# Autodesk Inventor assembly: アーム3
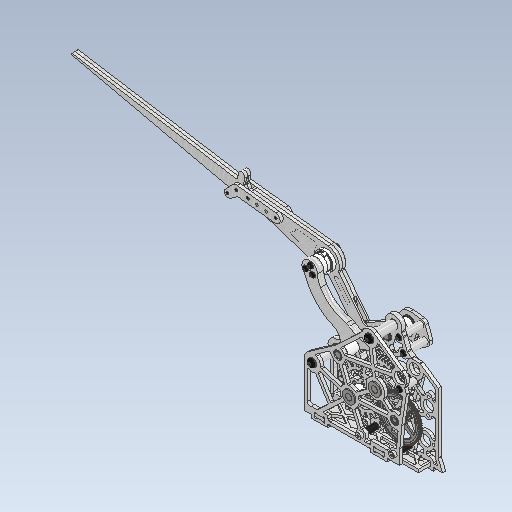
[picture p0: Inventor's stored thumbnail of the model, 512x512]
Saved by Autodesk Inventor 2020.3 (Build 243373000, 373)
## iProperties
Created: 2020-03-16
Part Number: アーム3
Document SubType Name: Assembly
Designer: aoyam
Mass: 278.23 g
Surface Area: 1026.87 cm^2
Volume: 86.6022 cm^3
Density: 3.21274 g/cm^3
Author: aoyam
## Documents named in this file (55)
- C:\Users\aoyam\Desktop\SRDC_local\Inventor\二年機\Geminiβ\腕\アーム3.iam
- C:\Users\aoyam\Desktop\SRDC_local\Inventor\二年機\Geminiβ\腕\アーム用初段.iam
- C:\Users\aoyam\Desktop\SRDC_local\Inventor\二年機\Geminiβ\腕\アーム用2段.iam
- C:\Users\aoyam\Desktop\SRDC_local\Inventor\二年機\Geminiβ\腕\アーム用3段.iam
- C:\Users\aoyam\Desktop\SRDC_local\Inventor\二年機\Geminiβ\腕\モーターマウント改.ipt
- C:\Users\aoyam\Desktop\SRDC_local\Inventor\二年機\Geminiβ\腕\アームフレーム改二.ipt
- C:\Users\aoyam\Desktop\SRDC_local\Inventor\二年機\Geminiβ\汎用部品\ベアリングHd6-D12-B4.ipt
- C:\Users\aoyam\Desktop\SRDC_local\Inventor\二年機\Geminiβ\汎用部品\ベアリングd4D8B3F.ipt
- C:\Users\aoyam\Desktop\SRDC_local\Inventor\二年機\Geminiβ\汎用部品\スペーサー中空M6L3アルミ自作.ipt
- C:\Users\aoyam\Desktop\SRDC_local\Inventor\二年機\Geminiβ\腕\アームギアフレーム最内2.ipt
- C:\Users\aoyam\Desktop\SRDC_local\Inventor\二年機\Geminiβ\腕\駆動軸.ipt
- C:\Users\aoyam\Desktop\SRDC_local\Inventor\二年機\Geminiβ\汎用部品\オイレスFd6D8L3.ipt
- C:\Users\aoyam\Desktop\SRDC_local\Inventor\二年機\Geminiβ\汎用部品\平行ピンD6L28.ipt
- C:\Users\aoyam\Desktop\SRDC_local\Inventor\二年機\Geminiβ\汎用部品\ワッシャD8d6m0.5.ipt
- C:\Users\aoyam\Desktop\SRDC_local\Inventor\二年機\Geminiβ\汎用部品\ワッシャD7d4m0.5.ipt
- C:\Users\aoyam\Desktop\SRDC_local\Inventor\二年機\Geminiβ\汎用部品\スペーサー中空M6L5樹脂.ipt
- C:\Users\aoyam\Desktop\SRDC_local\Inventor\二年機\Geminiβ\汎用部品\スペーサー中空M6L8樹脂.ipt
- C:\Users\aoyam\Desktop\SRDC_local\Inventor\二年機\Geminiβ\汎用部品\平行ピンD4L18.ipt
- C:\Users\aoyam\Desktop\SRDC_local\Inventor\二年機\Geminiβ\汎用部品\スペーサーM3L6アルミ .ipt
- C:\Users\aoyam\Desktop\SRDC_local\Inventor\二年機\Geminiβ\汎用部品\スペーサーM3L12アルミ.ipt
- C:\Users\aoyam\Desktop\SRDC_local\Inventor\二年機\Geminiβ\腕\アーム揺動節test.ipt
- C:\Users\aoyam\Desktop\SRDC_local\Inventor\二年機\Geminiβ\腕\アーム中間節test.ipt
- C:\Users\aoyam\Desktop\SRDC_local\Inventor\二年機\Geminiβ\汎用部品\オイレスFd6D8L6.ipt
- C:\Users\aoyam\Desktop\SRDC_local\Inventor\二年機\Geminiβ\腕\アームカムAL.ipt
- C:\Users\aoyam\Desktop\SRDC_local\Inventor\二年機\Geminiβ\腕\アーム中間その弐.ipt
- C:\Users\aoyam\Desktop\SRDC_local\Inventor\二年機\Geminiβ\汎用部品\ネジボタンM3L25.ipt
- C:\Users\aoyam\Desktop\SRDC_local\Inventor\二年機\Geminiβ\汎用部品\ネジボタンM3L6.ipt
- C:\Users\aoyam\Desktop\SRDC_local\Inventor\二年機\Geminiβ\汎用部品\オイレスF外径16内径14L9.ipt
- C:\Users\aoyam\Desktop\SRDC_local\Inventor\二年機\Geminiβ\汎用部品\ネジボタンM3L14.ipt
- C:\Users\aoyam\Desktop\SRDC_local\Inventor\二年機\Geminiβ\汎用部品\ネジボタンM4L6.ipt
- C:\Users\aoyam\Desktop\SRDC_local\Inventor\二年機\Geminiβ\腕\アーム揺動節抑え.ipt
- C:\Users\aoyam\Desktop\SRDC_local\Inventor\二年機\Geminiβ\汎用部品\スペーサーM3L18アルミ.ipt
- C:\Users\aoyam\Desktop\SRDC_local\Inventor\二年機\Geminiβ\腕\アーム底板.ipt
- C:\Users\aoyam\Desktop\SRDC_local\Inventor\二年機\Geminiβ\腕\アーム先端.iam
- C:\Users\aoyam\Desktop\SRDC_local\Inventor\二年機\Geminiβ\汎用部品\オイレス外径8内径6L3.ipt
- C:\Users\aoyam\Desktop\SRDC_local\Inventor\二年機\Geminiβ\汎用部品\スペーサーM3L12樹脂.ipt
- C:\Users\aoyam\Desktop\SRDC_local\Inventor\二年機\Geminiβ\汎用部品\スペーサーM3L6樹脂.ipt
- C:\Users\aoyam\Desktop\SRDC_local\Inventor\二年機\Geminiβ\汎用部品\平行ピンD6L30Dcut.ipt
- C:\Users\aoyam\Desktop\SRDC_local\Inventor\二年機\Geminiβ\汎用部品\電子機器類\RDC506018A\RDC506018A.ipt
- C:\Users\aoyam\Desktop\SRDC_local\Inventor\二年機\Geminiβ\汎用部品\ネジボタンM2L6.ipt
- C:\Users\aoyam\Desktop\SRDC_local\Inventor\二年機\Geminiβ\腕\アームカムD14.ipt
- C:\Users\aoyam\Desktop\SRDC_local\Inventor\二年機\Geminiβ\腕\アームカムD15t4.ipt
- C:\Users\aoyam\Desktop\SRDC_local\Inventor\二年機\Geminiβ\腕\アームカムFD18t4.ipt
- C:\Users\aoyam\Desktop\SRDC_local\Inventor\二年機\Geminiβ\腕\アームカムD18.ipt
- C:\Users\aoyam\Desktop\SRDC_local\Inventor\二年機\Geminiβ\汎用部品\スペーサー中空M6L2.5樹脂自作.ipt
- C:\Users\aoyam\Desktop\SRDC_local\Inventor\二年機\Geminiβ\汎用部品\スペーサーM4L21アルミ.ipt
- C:\Users\aoyam\Desktop\SRDC_local\Inventor\二年機\Geminiβ\汎用部品\ネジアルミM3L6.ipt
- C:\Users\aoyam\Desktop\SRDC_local\Inventor\二年機\Geminiβ\汎用部品\スペーサー中空M6L12樹脂.ipt
- C:\Users\aoyam\Desktop\SRDC_local\Inventor\二年機\Geminiβ\汎用部品\スペーサー中空M6L6樹脂.ipt
- C:\Users\aoyam\Desktop\SRDC_local\Inventor\二年機\インナー4層丙弐型\アーム\アーム3\AIP\FEA\d76wgh76o.fins
- C:\Users\aoyam\Desktop\SRDC_local\Inventor\二年機\インナー4層丙弐型\アーム\アーム3\AIP\FEA\d76wgh76o.fsat
- C:\Users\aoyam\Desktop\SRDC_local\Inventor\二年機\インナー4層丙弐型\アーム\アーム3\AIP\FEA\d76wgh76o.ftes
- C:\Users\aoyam\Desktop\SRDC_local\Inventor\二年機\インナー4層丙弐型\アーム\アーム3\AIP\FEA\d76wgh77k.fwiz
- C:\Users\aoyam\Desktop\SRDC_local\Inventor\二年機\インナー4層丙弐型\アーム\アーム3\AIP\FEA\d76wgh8o0.fmsh
- C:\Users\aoyam\Desktop\SRDC_local\Inventor\二年機\インナー4層丙弐型\アーム\アーム3\AIP\FEA\d76wgh8ow.fres
## Components (92 placed, 48 different names)
1. アーム用初段:1 [sub-assembly] — メイト:4, メイト:16, 挿入:204
2. アーム用2段:1 [sub-assembly] — メイト:4, メイト:6, メイト:21, メイト:27, 挿入:16, 挿入:31, 挿入:151
3. アーム用3段:1 [sub-assembly] — メイト:6, メイト:21, メイト:28, 挿入:41
4. モーターマウント改:1 — メイト:16, メイト:26, 挿入:17, メイト:30, 挿入:47, 挿入:109, メイト:73, 挿入:165, 挿入:166, 挿入:212, 挿入:213, 挿入:214, 挿入:216
5. アームフレーム改二:1 — メイト:26, メイト:27, メイト:28, 挿入:12, 挿入:13, 挿入:14, 挿入:32, 挿入:46, 挿入:135, メイト:74, 挿入:162, 挿入:208, 挿入:209, 挿入:211, 挿入:219
6. ベアリングHd6-D12-B4:1 — 挿入:13, 挿入:27
7. ベアリングd4D8B3F:1 — 挿入:12, 挿入:36, 挿入:42
8. ベアリングHd6-D12-B4:3 — 挿入:14, 挿入:28, 挿入:33
9. スペーサー中空M6L3アルミ自作:1 — 挿入:16
10. ベアリングd4D8B3F:2 — 挿入:17, 挿入:37
11. アームギアフレーム最内2:1 — メイト:30, 挿入:19, 挿入:20, 挿入:35, メイト:32, 挿入:105, 挿入:107, 挿入:110, 挿入:123, 挿入:126, メイト:69, メイト:70, メイト:71, 挿入:143, 挿入:144, 挿入:145, 挿入:150, メイト:72, 挿入:172, 挿入:173, 挿入:210, 挿入:215, 挿入:222, 角度:2, 挿入:227, 挿入:228
12. ベアリングHd6-D12-B4:4 — 挿入:19, 挿入:30, メイト:54
13. ベアリングHd6-D12-B4:5 — 挿入:20
14. 駆動軸:1 — 挿入:167, 挿入:168, 挿入:169, 挿入:201, 挿入:217, 挿入:221
15. オイレスFd6D8L3:1 — 挿入:219, 挿入:220
16. 平行ピンD6L28:1 — 挿入:27, メイト:54
17. 平行ピンD6L28:2 — 挿入:28
18. ワッシャD8d6m0.5:1 — 挿入:151
19. ワッシャD8d6m0.5:2 — 挿入:30, 挿入:39
20. ワッシャD8d6m0.5:3 — 挿入:31
21. ワッシャD8d6m0.5:4 — 挿入:32
22. ワッシャD8d6m0.5:5 — 挿入:33
23. ワッシャD8d6m0.5:7 — 挿入:35, 挿入:207
24. ワッシャD7d4m0.5:2 — 挿入:37, 挿入:205
25. ワッシャD7d4m0.5:3 — 挿入:36, 挿入:204
26. スペーサー中空M6L5樹脂:1 — 挿入:39
27. スペーサー中空M6L8樹脂:1 — 挿入:41
28. 平行ピンD4L18:1 — 挿入:42
29. スペーサーM3L12アルミ:2 — 挿入:46
30. スペーサーM3L6アルミ :2 — 挿入:47, 挿入:123
31. アーム揺動節test:1 — メイト:32, 挿入:122, 挿入:218
32. アーム中間節test:1 — 挿入:120, メイト:53, 挿入:158, 挿入:203
33. オイレスFd6D8L6:1 — 挿入:222, 挿入:223, 挿入:224
34. アームカムAL:1 — 挿入:194, 挿入:195, 挿入:196, 挿入:197, 挿入:200
35. アーム中間その弐:1 — 挿入:120, メイト:53, 挿入:122, 挿入:159, 挿入:189, メイト:84, 挿入:198
36. オイレスFd6D8L6:2 — 挿入:221, 挿入:226
37. オイレスF外径16内径14L9:1 — 挿入:197, 挿入:198, メイト:86, メイト:87
38. スペーサーM3L6アルミ :3 — 挿入:105
39. ネジボタンM3L14:1 — 挿入:107
40. ネジボタンM3L6:4 — 挿入:212
41. ネジボタンM3L6:5 — 挿入:109
42. ネジボタンM3L6:6 — 挿入:110
43. ネジボタンM3L6:7 — 挿入:211
44. ネジボタンM4L6:1 — 挿入:162
45. ネジボタンM4L6:2 — 挿入:126
46. ネジボタンM4L6:3 — 挿入:150
47. ネジボタンM4L6:4 — 挿入:135
48. オイレスFd6D8L6:3 — 挿入:225
49. アーム揺動節抑え:1 — メイト:69, メイト:70, メイト:71, 挿入:140, 挿入:141, 挿入:142, 挿入:146, 挿入:147, 挿入:148
50. スペーサーM3L18アルミ:1 — 挿入:140
51. スペーサーM3L18アルミ:2 — 挿入:141
52. スペーサーM3L18アルミ:3 — 挿入:142, 挿入:227
53. ネジボタンM3L6:16 — 挿入:143
54. ネジボタンM3L6:17 — 挿入:144
55. ネジボタンM3L6:18 — 挿入:145
56. ネジボタンM3L6:19 — 挿入:146
57. ネジボタンM3L6:20 — 挿入:147
58. ネジボタンM3L6:21 — 挿入:148
59. アーム底板:1 — メイト:72, メイト:73, メイト:74
60. アーム先端:1 [sub-assembly] — 挿入:189, メイト:84
61. オイレス外径8内径6L3:1 — 挿入:158
62. ネジボタンM3L6:22 — 挿入:159
63. スペーサーM3L12樹脂:1 — 挿入:165
64. スペーサーM3L12樹脂:2 — 挿入:166
65. スペーサーM3L6樹脂:1 — 挿入:228
66. ネジボタンM3L25:1 — 挿入:168, 挿入:196
67. ネジボタンM3L25:2 — 挿入:167, 挿入:195
68. ネジボタンM3L25:3 — 挿入:169, 挿入:194, メイト:88
69. 平行ピンD6L30Dcut:1 — 挿入:171, 角度:1, 挿入:226
70. RDC506018A:1 — 挿入:171, 角度:1, 角度:2
71. ネジボタンM2L6:1 — 挿入:172
72. ネジボタンM2L6:2 — 挿入:173
73. 平行ピンD6L28:3 — 挿入:224
74. アームカムD14:1 — 挿入:199, メイト:85, メイト:86, 挿入:202
75. アームカムD14:2 — 挿入:199, メイト:85, 挿入:200
76. アームカムD15t4:1 — 挿入:201, メイト:87
77. アームカムFD18t4:1 — 挿入:202, メイト:88
78. アームカムD18:1 — 挿入:203
79. スペーサー中空M6L2.5樹脂自作:1 — 挿入:205
80. ワッシャD8d6m0.5:8 — 挿入:206
81. ワッシャD8d6m0.5:9 — 挿入:206, 挿入:207
82. スペーサーM4L21アルミ:1 — 挿入:208, 挿入:210
83. スペーサーM4L21アルミ:2 — 挿入:209
84. ネジアルミM3L6:1
85. ネジアルミM3L6:2
86. ネジアルミM3L6:3 — 挿入:214
87. ネジアルミM3L6:4 — 挿入:213
88. ネジアルミM3L6:5 — 挿入:216
89. ネジアルミM3L6:6 — 挿入:215
90. スペーサー中空M6L12樹脂:1 — 挿入:217, 挿入:220
91. スペーサー中空M6L6樹脂:1 — 挿入:218, 挿入:225
92. スペーサー中空M6L6樹脂:2 — 挿入:223
## Relationships (112: Insert 88, Mate 22, Angle 2)
- メイト:4 [Mate] (0.5 mm): アーム用初段:1 ↔ アーム用2段:1
- メイト:6 [Mate] (0.5 mm): アーム用2段:1 ↔ アーム用3段:1
- メイト:16 [Mate]: アーム用初段:1 ↔ モーターマウント改:1
- メイト:21 [Mate] (0.5 mm): アーム用2段:1 ↔ アーム用3段:1
- メイト:26 [Mate]: モーターマウント改:1 ↔ アームフレーム改二:1
- メイト:27 [Mate]: アーム用2段:1 ↔ アームフレーム改二:1
- メイト:28 [Mate]: アーム用3段:1 ↔ アームフレーム改二:1
- 挿入:12 [Insert]: アームフレーム改二:1 ↔ ベアリングd4D8B3F:1
- 挿入:13 [Insert]: アームフレーム改二:1 ↔ ベアリングHd6-D12-B4:1
- 挿入:14 [Insert]: アームフレーム改二:1 ↔ ベアリングHd6-D12-B4:3
- 挿入:16 [Insert] (0.5 mm): アーム用2段:1 ↔ スペーサー中空M6L3アルミ自作:1
- 挿入:17 [Insert]: モーターマウント改:1 ↔ ベアリングd4D8B3F:2
- メイト:30 [Mate]: モーターマウント改:1 ↔ アームギアフレーム最内2:1
- 挿入:19 [Insert]: アームギアフレーム最内2:1 ↔ ベアリングHd6-D12-B4:4
- 挿入:20 [Insert]: アームギアフレーム最内2:1 ↔ ベアリングHd6-D12-B4:5
- 挿入:27 [Insert]: ベアリングHd6-D12-B4:1 ↔ 平行ピンD6L28:1
- 挿入:28 [Insert]: ベアリングHd6-D12-B4:3 ↔ 平行ピンD6L28:2
- 挿入:30 [Insert]: ベアリングHd6-D12-B4:4 ↔ ワッシャD8d6m0.5:2
- 挿入:31 [Insert]: アーム用2段:1 ↔ ワッシャD8d6m0.5:3
- 挿入:32 [Insert]: アームフレーム改二:1 ↔ ワッシャD8d6m0.5:4
- 挿入:33 [Insert]: ベアリングHd6-D12-B4:3 ↔ ワッシャD8d6m0.5:5
- 挿入:35 [Insert]: アームギアフレーム最内2:1 ↔ ワッシャD8d6m0.5:7
- 挿入:36 [Insert]: ベアリングd4D8B3F:1 ↔ ワッシャD7d4m0.5:3
- 挿入:37 [Insert]: ベアリングd4D8B3F:2 ↔ ワッシャD7d4m0.5:2
- 挿入:39 [Insert]: ワッシャD8d6m0.5:2 ↔ スペーサー中空M6L5樹脂:1
- 挿入:41 [Insert]: アーム用3段:1 ↔ スペーサー中空M6L8樹脂:1
- 挿入:42 [Insert]: ベアリングd4D8B3F:1 ↔ 平行ピンD4L18:1
- 挿入:46 [Insert]: アームフレーム改二:1 ↔ スペーサーM3L12アルミ:2
- 挿入:47 [Insert]: モーターマウント改:1 ↔ スペーサーM3L6アルミ :2
- メイト:32 [Mate]: アームギアフレーム最内2:1 ↔ アーム揺動節test:1
- 挿入:105 [Insert]: アームギアフレーム最内2:1 ↔ スペーサーM3L6アルミ :3
- 挿入:107 [Insert]: アームギアフレーム最内2:1 ↔ ネジボタンM3L14:1
- 挿入:109 [Insert]: モーターマウント改:1 ↔ ネジボタンM3L6:5
- 挿入:110 [Insert]: アームギアフレーム最内2:1 ↔ ネジボタンM3L6:6
- 挿入:120 [Insert]: アーム中間節test:1 ↔ アーム中間その弐:1
- メイト:53 [Mate]: アーム中間節test:1 ↔ アーム中間その弐:1
- 挿入:122 [Insert]: アーム揺動節test:1 ↔ アーム中間その弐:1
- 挿入:123 [Insert]: アームギアフレーム最内2:1 ↔ スペーサーM3L6アルミ :2
- メイト:54 [Mate]: ベアリングHd6-D12-B4:4 ↔ 平行ピンD6L28:1
- 挿入:126 [Insert]: アームギアフレーム最内2:1 ↔ ネジボタンM4L6:2
- 挿入:135 [Insert]: アームフレーム改二:1 ↔ ネジボタンM4L6:4
- メイト:69 [Mate]: アームギアフレーム最内2:1 ↔ アーム揺動節抑え:1
- メイト:70 [Mate]: アームギアフレーム最内2:1 ↔ アーム揺動節抑え:1
- メイト:71 [Mate]: アームギアフレーム最内2:1 ↔ アーム揺動節抑え:1
- 挿入:140 [Insert]: アーム揺動節抑え:1 ↔ スペーサーM3L18アルミ:1
- 挿入:141 [Insert]: アーム揺動節抑え:1 ↔ スペーサーM3L18アルミ:2
- 挿入:142 [Insert]: アーム揺動節抑え:1 ↔ スペーサーM3L18アルミ:3
- 挿入:143 [Insert]: アームギアフレーム最内2:1 ↔ ネジボタンM3L6:16
- 挿入:144 [Insert]: アームギアフレーム最内2:1 ↔ ネジボタンM3L6:17
- 挿入:145 [Insert]: アームギアフレーム最内2:1 ↔ ネジボタンM3L6:18
- 挿入:146 [Insert]: アーム揺動節抑え:1 ↔ ネジボタンM3L6:19
- 挿入:147 [Insert]: アーム揺動節抑え:1 ↔ ネジボタンM3L6:20
- 挿入:148 [Insert]: アーム揺動節抑え:1 ↔ ネジボタンM3L6:21
- 挿入:150 [Insert]: アームギアフレーム最内2:1 ↔ ネジボタンM4L6:3
- 挿入:151 [Insert]: アーム用2段:1 ↔ ワッシャD8d6m0.5:1
- メイト:72 [Mate]: アームギアフレーム最内2:1 ↔ アーム底板:1
- メイト:73 [Mate]: モーターマウント改:1 ↔ アーム底板:1
- メイト:74 [Mate]: アームフレーム改二:1 ↔ アーム底板:1
- 挿入:158 [Insert]: アーム中間節test:1 ↔ オイレス外径8内径6L3:1
- 挿入:159 [Insert]: アーム中間その弐:1 ↔ ネジボタンM3L6:22
- 挿入:162 [Insert]: アームフレーム改二:1 ↔ ネジボタンM4L6:1
- 挿入:165 [Insert]: モーターマウント改:1 ↔ スペーサーM3L12樹脂:1
- 挿入:166 [Insert]: モーターマウント改:1 ↔ スペーサーM3L12樹脂:2
- 挿入:167 [Insert]: 駆動軸:1 ↔ ネジボタンM3L25:2
- 挿入:168 [Insert]: 駆動軸:1 ↔ ネジボタンM3L25:1
- 挿入:169 [Insert]: 駆動軸:1 ↔ ネジボタンM3L25:3
- 挿入:171 [Insert]: 平行ピンD6L30Dcut:1 ↔ RDC506018A:1
- 角度:1 [Angle] (180 deg): 平行ピンD6L30Dcut:1 ↔ RDC506018A:1
- 挿入:172 [Insert] (3.1 mm): アームギアフレーム最内2:1 ↔ ネジボタンM2L6:1
- 挿入:173 [Insert] (3.1 mm): アームギアフレーム最内2:1 ↔ ネジボタンM2L6:2
- 挿入:189 [Insert]: アーム中間その弐:1 ↔ アーム先端:1
- メイト:84 [Mate]: アーム中間その弐:1 ↔ アーム先端:1
- 挿入:194 [Insert]: アームカムAL:1 ↔ ネジボタンM3L25:3
- 挿入:195 [Insert]: アームカムAL:1 ↔ ネジボタンM3L25:2
- 挿入:196 [Insert]: アームカムAL:1 ↔ ネジボタンM3L25:1
- 挿入:197 [Insert]: アームカムAL:1 ↔ オイレスF外径16内径14L9:1
- 挿入:198 [Insert]: アーム中間その弐:1 ↔ オイレスF外径16内径14L9:1
- 挿入:199 [Insert]: アームカムD14:1 ↔ アームカムD14:2
- メイト:85 [Mate]: アームカムD14:1 ↔ アームカムD14:2
- 挿入:200 [Insert]: アームカムAL:1 ↔ アームカムD14:2
- メイト:86 [Mate]: オイレスF外径16内径14L9:1 ↔ アームカムD14:1
- 挿入:201 [Insert]: 駆動軸:1 ↔ アームカムD15t4:1
- メイト:87 [Mate]: オイレスF外径16内径14L9:1 ↔ アームカムD15t4:1
- 挿入:202 [Insert]: アームカムD14:1 ↔ アームカムFD18t4:1
- メイト:88 [Mate]: ネジボタンM3L25:3 ↔ アームカムFD18t4:1
- 挿入:203 [Insert]: アーム中間節test:1 ↔ アームカムD18:1
- 挿入:204 [Insert]: アーム用初段:1 ↔ ワッシャD7d4m0.5:3
- 挿入:205 [Insert]: ワッシャD7d4m0.5:2 ↔ スペーサー中空M6L2.5樹脂自作:1
- 挿入:206 [Insert]: ワッシャD8d6m0.5:8 ↔ ワッシャD8d6m0.5:9
- 挿入:207 [Insert]: ワッシャD8d6m0.5:7 ↔ ワッシャD8d6m0.5:9
- 挿入:208 [Insert]: アームフレーム改二:1 ↔ スペーサーM4L21アルミ:1
- 挿入:209 [Insert]: アームフレーム改二:1 ↔ スペーサーM4L21アルミ:2
- 挿入:210 [Insert]: アームギアフレーム最内2:1 ↔ スペーサーM4L21アルミ:1
- 挿入:211 [Insert]: アームフレーム改二:1 ↔ ネジボタンM3L6:7
- 挿入:212 [Insert]: モーターマウント改:1 ↔ ネジボタンM3L6:4
- 挿入:213 [Insert]: モーターマウント改:1 ↔ ネジアルミM3L6:4
- 挿入:214 [Insert]: モーターマウント改:1 ↔ ネジアルミM3L6:3
- 挿入:215 [Insert]: アームギアフレーム最内2:1 ↔ ネジアルミM3L6:6
- 挿入:216 [Insert]: モーターマウント改:1 ↔ ネジアルミM3L6:5
- 挿入:217 [Insert]: 駆動軸:1 ↔ スペーサー中空M6L12樹脂:1
- 挿入:218 [Insert]: アーム揺動節test:1 ↔ スペーサー中空M6L6樹脂:1
- 挿入:219 [Insert]: アームフレーム改二:1 ↔ オイレスFd6D8L3:1
- 挿入:220 [Insert]: オイレスFd6D8L3:1 ↔ スペーサー中空M6L12樹脂:1
- 挿入:221 [Insert]: 駆動軸:1 ↔ オイレスFd6D8L6:2
- 挿入:222 [Insert]: アームギアフレーム最内2:1 ↔ オイレスFd6D8L6:1
- 挿入:223 [Insert]: オイレスFd6D8L6:1 ↔ スペーサー中空M6L6樹脂:2
- 挿入:224 [Insert] (-0.5 mm): オイレスFd6D8L6:1 ↔ 平行ピンD6L28:3
- 挿入:225 [Insert]: オイレスFd6D8L6:3 ↔ スペーサー中空M6L6樹脂:1
- 挿入:226 [Insert]: オイレスFd6D8L6:2 ↔ 平行ピンD6L30Dcut:1
- 角度:2 [Angle] (0 deg): アームギアフレーム最内2:1 ↔ RDC506018A:1
- 挿入:227 [Insert]: アームギアフレーム最内2:1 ↔ スペーサーM3L18アルミ:3
- 挿入:228 [Insert]: アームギアフレーム最内2:1 ↔ スペーサーM3L6樹脂:1
## Named parameters: sa_0 = 3200
note: some values were not read from the file. Shown as the stored number, unit unknown: "sa_0".
